# Autodesk Inventor assembly: 四方轴套 正 头洞
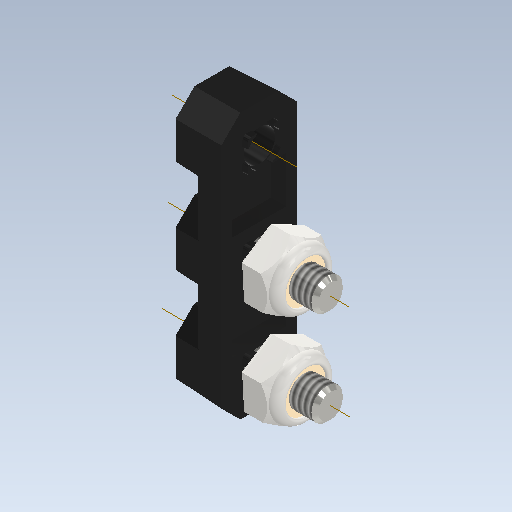
[picture p0: Inventor's stored thumbnail of the model, 512x512]
Saved by Autodesk Inventor 2020 (Build 240168000, 168)
## iProperties
Created: 2019-05-29
Part Number: 四方轴套 正 头洞
Document SubType Name: Assembly
Designer: aresp
Mass: 19.0752 g
Surface Area: 27.5884 cm^2
Volume: 2.44333 cm^3
Density: 7.80703 g/cm^3
Author: aresp
## Documents named in this file (3)
- C:\Users\hp\Documents\Vault\ncrCadLib\轴相关\细轴配套\四方轴套 正 头洞.iam
- C:\Users\hp\Documents\Vault\ncrCadLib\轴相关\细轴配套\零件\细轴四方轴承.ipt
- C:\Users\hp\Documents\Vault\ncrCadLib\轴相关\粗轴配套\零件\四号螺丝+防滑.iam
## Components (3 placed, 2 different names)
1. 细轴四方轴承:1 — 配合:3, 配合:4
2. 四号螺丝+防滑:1 [sub-assembly] — 配合:3
3. 四号螺丝+防滑:2 [sub-assembly] — 配合:4
## Component patterns: (2 elements, first: 四号螺丝+防滑:1)
## Relationships (2: Mate 2)
- 配合:3 [Mate]: 细轴四方轴承:1 ↔ 四号螺丝+防滑:1
- 配合:4 [Mate]: 细轴四方轴承:1 ↔ 四号螺丝+防滑:2
